# Autodesk Inventor assembly: Láser_cavidad_piezo_chico
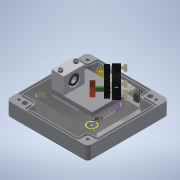
[picture p0: Inventor's stored thumbnail of the model, 180x180]
Saved by Autodesk Inventor 2022.2 (Build 262287010, 287A)
## iProperties
Created: 2018-04-02
Part Number: Láser_cavidad_piezo_chico
Document SubType Name: Assembly
Designer: Hogar
Author: Hogar
## Documents named in this file (10)
- E:\pixki\OCR\Designs\lasers\ECDL OCR\Láser_cavidad_piezo_chico.iam
- E:\pixki\OCR\Designs\lasers\ECDL OCR\5500-37 LID.ipt
- E:\pixki\OCR\Designs\lasers\ECDL OCR\ECDL.iam
- E:\pixki\OCR\Designs\lasers\ECDL OCR\5500-37 Box.ipt
- E:\pixki\OCR\Designs\lasers\ECDL OCR\Placa base.ipt
- E:\pixki\OCR\Designs\lasers\ECDL OCR\Components\743209004.ipt
- E:\pixki\OCR\Designs\lasers\ECDL OCR\Components\717811000.ipt
- E:\pixki\OCR\Designs\lasers\ECDL OCR\Components\132203.ipt
- E:\pixki\OCR\Designs\lasers\ECDL OCR\Components\934MD.ipt
- E:\pixki\OCR\Designs\lasers\ECDL OCR\Components\130WCP.ipt
## Components (10 placed, 9 different names)
1. 5500-37 LID:1 — Mate:1, Flush:1, Mate:4, Mate:6, Mate:7, Mate:8, Mate:9, Mate:10, Mate:11, Mate:12, Mate:13, Mate:14, Mate:15, Flush:4, Mate:16, Flush:5, Mate:17, Mate:18, Mate:19, Mate:20, Mate:22, Mate:23
2. Placa base:1 — Mate:4, Mate:5, Flush:3, Mate:22, Mate:23
3. ECDL:1 [sub-assembly] — Mate:5
4. 5500-37 Box:1 — Mate:6, Mate:7, Mate:8, Flush:2
5. 743209004:1 — Mate:9, Mate:10, Mate:11, Angle:1, Angle:2, Angle:3, Flush:7, Flush:8
6. 717811000:3 — Mate:12, Mate:14
7. 717811000:4 — Mate:13, Mate:15
8. 132203:1 — Mate:16, Flush:5, Angle:1, Flush:10, Flush:11
9. 934MD:1 — Mate:17, Mate:18, Angle:2
10. 130WCP:1 — Mate:19, Mate:20, Angle:3, Flush:6, Flush:9
## Relationships (34: Mate 20, Flush 11, Angle 3)
- Mate:1: 5500-37 LID:1
- Flush:1 (-74.8 mm): 5500-37 LID:1
- Mate:4: 5500-37 LID:1 ↔ Placa base:1
- Mate:5: Placa base:1 ↔ ECDL:1
- Mate:6: 5500-37 LID:1 ↔ 5500-37 Box:1
- Mate:7: 5500-37 LID:1 ↔ 5500-37 Box:1
- Mate:8: 5500-37 LID:1 ↔ 5500-37 Box:1
- Flush:2 (72.7 mm): 5500-37 Box:1
- Flush:3 (-40 mm): Placa base:1
- Mate:9: 5500-37 LID:1 ↔ 743209004:1
- Mate:10 (3.11 mm): 5500-37 LID:1 ↔ 743209004:1
- Mate:11 (2.985 mm): 5500-37 LID:1 ↔ 743209004:1
- Mate:12: 5500-37 LID:1 ↔ 717811000:3
- Mate:13: 5500-37 LID:1 ↔ 717811000:4
- Mate:14: 5500-37 LID:1 ↔ 717811000:3
- Mate:15: 5500-37 LID:1 ↔ 717811000:4
- Flush:4 (24.03 mm): 5500-37 LID:1
- Mate:16: 5500-37 LID:1 ↔ 132203:1
- Flush:5: 5500-37 LID:1 ↔ 132203:1
- Angle:1 (270 deg): 743209004:1 ↔ 132203:1
- Mate:17: 5500-37 LID:1 ↔ 934MD:1
- Mate:18: 5500-37 LID:1 ↔ 934MD:1
- Angle:2 (270 deg): 743209004:1 ↔ 934MD:1
- Mate:19: 5500-37 LID:1 ↔ 130WCP:1
- Mate:20: 5500-37 LID:1 ↔ 130WCP:1
- Angle:3 (270 deg): 743209004:1 ↔ 130WCP:1
- Mate:22: 5500-37 LID:1 ↔ Placa base:1
- Mate:23: 5500-37 LID:1 ↔ Placa base:1
- Flush:6 (-0.25 mm): 130WCP:1
- Flush:7 (-0.25 mm): 743209004:1
- Flush:8 (-0.1525 mm): 743209004:1
- Flush:9 (-0.25 mm): 130WCP:1
- Flush:10 (0.51 mm): 132203:1
- Flush:11 (0.51 mm): 132203:1
